# Autodesk Inventor assembly: XL430-bracket
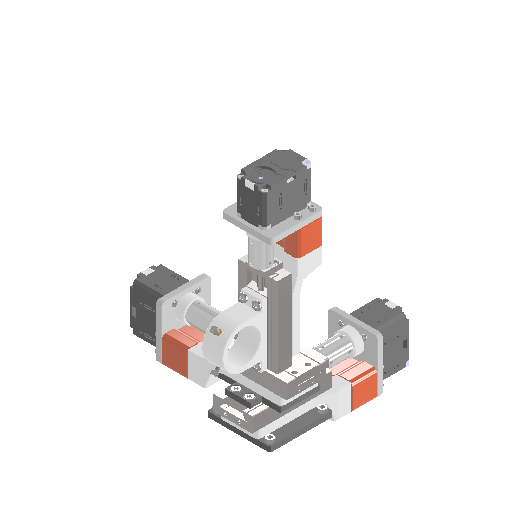
[picture p0: Inventor's stored thumbnail of the model, 512x512]
Saved by Autodesk Inventor 2026.2 (Build 302298000, 298)
## iProperties
Created: 2025-05-28
Part Number: XL430-bracket
Document SubType Name: Assembly
Designer: kuzmin
Mass: 1365.19 g
Surface Area: 1309.73 cm^2
Volume: 325.346 cm^3
Density: 4.19612 g/cm^3
Author: kuzmin
## Documents named in this file (12)
- D:\repos\PIHTI\LIBS\XL430-bracket.iam
- D:\repos\PIHTI\LIBS\TAS-20605L\TAS-60-09B.ipt
- D:\repos\PIHTI\LIBS\TAS-20605L\TAS-dovegroove.ipt
- D:\repos\PIHTI\LIBS\TAS-20605L\TAS-60XYZ-Y-slider.ipt
- D:\repos\PIHTI\LIBS\TAS-20605L\TAS-60XYZ-cross-plate.ipt
- D:\repos\PIHTI\LIBS\Motor-Bracket-with-inserts.iam
- D:\repos\PIHTI\ContentCenter\Fastners\M4x10-SHCS.ipt
- D:\repos\PIHTI\ContentCenter\Fastners\M4x12-Fillips-Countersink.ipt
- D:\repos\PIHTI\LIBS\TAS-20605L\TAS-60XYZ-mounting-plate.ipt
- D:\repos\PIHTI\ContentCenter\Fastners\M4-nut.ipt
- D:\repos\PIHTI\ContentCenter\Fastners\M4x10-fillips-round.ipt
- D:\repos\PIHTI\LIBS\lens-clamp-hsi.iam
## Components (32 placed, 11 different names)
1. TAS-60-09B:1 — メイト:4, フラッシュ:1, フラッシュ:7, フラッシュ:8
2. TAS-dovegroove:1 — メイト:4, フラッシュ:1, リジッド:3, フラッシュ:7, フラッシュ:8, リジッド:22
3. TAS-60-09B:2 — フラッシュ:3, メイト:9, フラッシュ:5, リジッド:31
4. TAS-dovegroove:2 — フラッシュ:3, メイト:9, フラッシュ:5, リジッド:23
5. TAS-dovegroove:3 — フラッシュ:2, メイト:8, フラッシュ:9, リジッド:25
6. TAS-60XYZ-Y-slider:1 — フラッシュ:2, メイト:8, リジッド:3, フラッシュ:9
7. TAS-60XYZ-cross-plate:1 — リジッド:27, リジッド:28, リジッド:29, リジッド:30, リジッド:26, リジッド:31
8. Motor-Bracket-with-inserts:1 [sub-assembly] — リジッド:22, 回転:7, 回転:8, 回転:9, 回転:10
9. Motor-Bracket-with-inserts:2 [sub-assembly] — リジッド:25, リジッド:26
10. Motor-Bracket-with-inserts:3 [sub-assembly] — リジッド:21, リジッド:23
11. TAS-60XYZ-mounting-plate:1 — リジッド:13, リジッド:14, リジッド:15, リジッド:16, リジッド:17, リジッド:18, リジッド:19, リジッド:20, リジッド:21
12. lens-clamp-hsi:1 [sub-assembly]
13. BS EN ISO 7045 H - Metric M4 x 10 - 4.8 - H:1
14. BS EN ISO 7045 H - Metric M4 x 10 - 4.8 - H:2
15. BS EN ISO 7045 H - Metric M4 x 10 - 4.8 - H:3
16. BS EN ISO 7045 H - Metric M4 x 10 - 4.8 - H:4
17. JIS B 1181 -finished Class 1 - Metric Class 1 -finishedM4:1 — リジッド:20
18. JIS B 1181 -finished Class 1 - Metric Class 1 -finishedM4:2 — リジッド:19
19. JIS B 1181 -finished Class 1 - Metric Class 1 -finishedM4:3 — リジッド:18
20. JIS B 1181 -finished Class 1 - Metric Class 1 -finishedM4:4 — リジッド:17
21. AS 1427 Z - Metric M4 x 12:5 — リジッド:14
22. AS 1427 Z - Metric M4 x 12:6 — リジッド:16
23. AS 1427 Z - Metric M4 x 12:7 — リジッド:15
24. AS 1427 Z - Metric M4 x 12:8 — リジッド:13
25. AS 1427 Z - Metric M4 x 12:1 — リジッド:29
26. AS 1427 Z - Metric M4 x 12:2 — リジッド:28
27. AS 1427 Z - Metric M4 x 12:3 — リジッド:27
28. AS 1427 Z - Metric M4 x 12:4 — リジッド:30
29. AS 1420 - Metric M4 x 10:1 — 回転:8
30. AS 1420 - Metric M4 x 10:2 — 回転:7
31. AS 1420 - Metric M4 x 10:3 — 回転:9
32. AS 1420 - Metric M4 x 10:4 — 回転:10
## Relationships (38: WeldJoint 24, Flush 7, RevoluteJoint 4, Mate 3)
- メイト:4 [Mate]: TAS-60-09B:1 ↔ TAS-dovegroove:1
- フラッシュ:1 [Flush]: TAS-60-09B:1 ↔ TAS-dovegroove:1
- フラッシュ:2 [Flush]: TAS-dovegroove:3 ↔ TAS-60XYZ-Y-slider:1
- メイト:8 [Mate]: TAS-dovegroove:3 ↔ TAS-60XYZ-Y-slider:1
- フラッシュ:3 [Flush]: TAS-60-09B:2 ↔ TAS-dovegroove:2
- メイト:9 [Mate]: TAS-60-09B:2 ↔ TAS-dovegroove:2
- リジッド:3 [WeldJoint]: TAS-dovegroove:1 ↔ TAS-60XYZ-Y-slider:1
- フラッシュ:5 [Flush]: TAS-60-09B:2 ↔ TAS-dovegroove:2
- フラッシュ:7 [Flush]: TAS-60-09B:1 ↔ TAS-dovegroove:1
- フラッシュ:8 [Flush]: TAS-60-09B:1 ↔ TAS-dovegroove:1
- フラッシュ:9 [Flush]: TAS-dovegroove:3 ↔ TAS-60XYZ-Y-slider:1
- リジッド:27 [WeldJoint]: TAS-60XYZ-cross-plate:1 ↔ AS 1427 Z - Metric M4 x 12:3
- リジッド:28 [WeldJoint]: TAS-60XYZ-cross-plate:1 ↔ AS 1427 Z - Metric M4 x 12:2
- リジッド:29 [WeldJoint]: TAS-60XYZ-cross-plate:1 ↔ AS 1427 Z - Metric M4 x 12:1
- リジッド:30 [WeldJoint]: TAS-60XYZ-cross-plate:1 ↔ AS 1427 Z - Metric M4 x 12:4
- リジッド:13 [WeldJoint]: TAS-60XYZ-mounting-plate:1 ↔ AS 1427 Z - Metric M4 x 12:8
- リジッド:14 [WeldJoint]: TAS-60XYZ-mounting-plate:1 ↔ AS 1427 Z - Metric M4 x 12:5
- リジッド:15 [WeldJoint]: TAS-60XYZ-mounting-plate:1 ↔ AS 1427 Z - Metric M4 x 12:7
- リジッド:16 [WeldJoint]: TAS-60XYZ-mounting-plate:1 ↔ AS 1427 Z - Metric M4 x 12:6
- リジッド:17 [WeldJoint]: TAS-60XYZ-mounting-plate:1 ↔ JIS B 1181 -finished Class 1 - Metric Class 1 -finishedM4:4
- リジッド:18 [WeldJoint]: TAS-60XYZ-mounting-plate:1 ↔ JIS B 1181 -finished Class 1 - Metric Class 1 -finishedM4:3
- リジッド:19 [WeldJoint]: TAS-60XYZ-mounting-plate:1 ↔ JIS B 1181 -finished Class 1 - Metric Class 1 -finishedM4:2
- リジッド:20 [WeldJoint]: TAS-60XYZ-mounting-plate:1 ↔ JIS B 1181 -finished Class 1 - Metric Class 1 -finishedM4:1
- リジッド:21 [WeldJoint]: Motor-Bracket-with-inserts:3 ↔ TAS-60XYZ-mounting-plate:1
- リジッド:22 [WeldJoint]: TAS-dovegroove:1 ↔ Motor-Bracket-with-inserts:1
- リジッド:23 [WeldJoint]: TAS-dovegroove:2 ↔ Motor-Bracket-with-inserts:3
- リジッド:25 [WeldJoint]: TAS-dovegroove:3 ↔ Motor-Bracket-with-inserts:2
- リジッド:26 [WeldJoint]: TAS-60XYZ-cross-plate:1 ↔ Motor-Bracket-with-inserts:2
- [WeldJoint]: TAS-60-09B:1 ↔ lens-clamp-hsi:1
- 回転:7 [RevoluteJoint]: Motor-Bracket-with-inserts:1 ↔ AS 1420 - Metric M4 x 10:2
- 回転:8 [RevoluteJoint]: Motor-Bracket-with-inserts:1 ↔ AS 1420 - Metric M4 x 10:1
- 回転:9 [RevoluteJoint]: Motor-Bracket-with-inserts:1 ↔ AS 1420 - Metric M4 x 10:3
- 回転:10 [RevoluteJoint]: Motor-Bracket-with-inserts:1 ↔ AS 1420 - Metric M4 x 10:4
- リジッド:31 [WeldJoint]: TAS-60-09B:2 ↔ TAS-60XYZ-cross-plate:1
- [WeldJoint]: lens-clamp-hsi:1 ↔ BS EN ISO 7045 H - Metric M4 x 10 - 4.8 - H:4
- [WeldJoint]: lens-clamp-hsi:1 ↔ BS EN ISO 7045 H - Metric M4 x 10 - 4.8 - H:2
- [WeldJoint]: lens-clamp-hsi:1 ↔ BS EN ISO 7045 H - Metric M4 x 10 - 4.8 - H:1
- [WeldJoint]: lens-clamp-hsi:1 ↔ BS EN ISO 7045 H - Metric M4 x 10 - 4.8 - H:3
